# Autodesk Inventor assembly: modularRICHTurntable
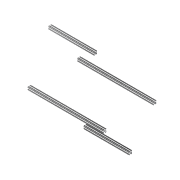
[picture p0: Inventor's stored thumbnail of the model, 180x180]
Saved by Autodesk Inventor 2018.2 (Build 222227000, 227)
## iProperties
Created: 2018-05-06
Part Number: modularRICHTurntable
Document SubType Name: Assembly
Designer: sawaiz
Author: sawaiz
## Documents named in this file (3)
- C:\Users\sawaiz\OneDrive\projects\modularRICHTurntable\modularRICHTurntable.iam
- C:\Users\sawaiz\OneDrive\projects\modularRICHFrame\frame\hfs5-2020Depth.ipt
- C:\Users\sawaiz\OneDrive\projects\modularRICHFrame\frame\hfs5-2020Width.ipt
## Components (4 placed, 2 different names)
1. hfs5-2020Depth:1 — Flush:1, Flush:2, Symmetry:1, Symmetry:2, Symmetry:3
2. hfs5-2020Depth:2 — Flush:1, Flush:2, Symmetry:1, Symmetry:2, Symmetry:3
3. hfs5-2020Width:1
4. hfs5-2020Width:2
## Relationships (5: Symmetry 3, Flush 2)
- Flush:1: hfs5-2020Depth:1 ↔ hfs5-2020Depth:2
- Flush:2: hfs5-2020Depth:1 ↔ hfs5-2020Depth:2
- Symmetry:1: hfs5-2020Depth:1 ↔ hfs5-2020Depth:2
- Symmetry:2: hfs5-2020Depth:1 ↔ hfs5-2020Depth:2
- Symmetry:3: hfs5-2020Depth:1 ↔ hfs5-2020Depth:2
